# Autodesk Inventor assembly: Drive Tube Assem
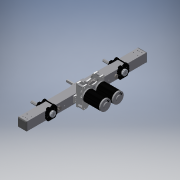
[picture p0: Inventor's stored thumbnail of the model, 180x180]
Saved by Autodesk Inventor 2019 (Build 230136000, 136)
## iProperties
Created: 2018-11-11
Part Number: Drive Tube Assem
Document SubType Name: Assembly
Designer: maste
Author: maste
## Documents named in this file (11)
- D:\Summer Drive Base V1\Summer Drivebase\Drive Tube Assem.iam
- D:\Summer Drive Base V1\Summer Drivebase\2x2 26in.ipt
- D:\Summer Drive Base V1\Summer Drivebase\Bearing Block Assem.iam
- D:\Summer Drive Base V1\Summer Drivebase\1in Spacer.ipt
- D:\Summer Drive Base V1\Summer Drivebase\0.0625in Spacer.ipt
- D:\Summer Drive Base V1\Summer Drivebase\36t_x_9mm_Wide_Double_Flange_Aluminum_Pulley_GT2_3mm_1_2_Hex_Bore_217-5873.ipt
- D:\Summer Drive Base V1\Summer Drivebase\Gearbox Assem.iam
- D:\Summer Drive Base V1\Summer Drivebase\Bearing Plate+Bearing.iam
- D:\Summer Drive Base V1\Summer Drivebase\0.125in Spacer.ipt
- D:\Summer Drive Base V1\Summer Drivebase\End Cap.ipt
- D:\Summer Drive Base V1\Summer Drivebase\217-3431-STEP.ipt
## Components (27 placed, 10 different names)
1. 2x2 26in:1 — Mate:1, Mate:2, Mate:3, Mate:4, Mate:5, Mate:6, Mate:27, Mate:28, Mate:29, Mate:30, Mate:31, Mate:32, Rotation:1, Mate:52, Mate:53, Mate:54, Mate:55, Mate:56, Mate:57, Mate:58, Mate:59, Rotation:2, Mate:60, Mate:61, Rotation:3
2. Bearing Block Assem:1 [sub-assembly] — Mate:4, Mate:5, Mate:6, Mate:7, Mate:8, Mate:9, Mate:14, Mate:17, Mate:18, Mate:20, Mate:21, Mate:43, Mate:44, Mate:45
3. Bearing Block Assem:2 [sub-assembly] — Mate:1, Mate:2, Mate:3, Mate:10, Mate:11, Mate:12, Mate:24, Mate:25, Mate:26, Mate:49, Mate:50, Mate:51
4. 1in Spacer:1 — Mate:10, Mate:11, Mate:12
5. 1in Spacer:2 — Mate:7, Mate:8, Mate:9, Mate:13, Mate:15
6. 0.0625in Spacer:1 — Mate:13, Mate:14, Mate:15, Mate:16
7. 0.0625in Spacer:2 — Mate:23, Flush:3, Flush:4
8. 36t_x_9mm_Wide_Double_Flange_Aluminum_Pulley_GT2_3mm_1_2_Hex_Bore_217-5873:1 — Mate:22, Flush:1, Flush:2, Mate:23, Flush:3, Flush:4
9. 36t_x_9mm_Wide_Double_Flange_Aluminum_Pulley_GT2_3mm_1_2_Hex_Bore_217-5873:2 — Mate:16, Mate:17, Mate:18, Mate:19
10. 0.0625in Spacer:3 — Mate:19, Mate:20, Mate:21
11. 0.0625in Spacer:4 — Mate:22, Flush:1, Flush:2, Mate:24, Mate:25, Mate:26
12. Gearbox Assem:1 [sub-assembly] — Mate:27, Mate:28, Mate:29, Mate:41, Mate:42, Mate:47, Mate:48
13. Bearing Plate+Bearing:1 [sub-assembly] — Mate:30, Mate:31, Mate:32, Rotation:1, Mate:40, Mate:46
14. 0.125in Spacer:1 — Mate:36, Flush:11, Flush:12, Mate:37, Flush:13, Flush:14
15. 0.125in Spacer:2 — Mate:35, Flush:9, Flush:10, Mate:36, Flush:11, Flush:12
16. 0.125in Spacer:3 — Mate:34, Flush:7, Flush:8, Mate:35, Flush:9, Flush:10
17. 36t_x_9mm_Wide_Double_Flange_Aluminum_Pulley_GT2_3mm_1_2_Hex_Bore_217-5873:3 — Mate:34, Flush:7, Flush:8, Mate:39, Flush:17, Flush:18
18. 36t_x_9mm_Wide_Double_Flange_Aluminum_Pulley_GT2_3mm_1_2_Hex_Bore_217-5873:4 — Mate:37, Flush:13, Flush:14, Mate:38, Flush:15, Flush:16
19. 0.125in Spacer:4 — Mate:39, Flush:17, Flush:18
20. 0.125in Spacer:5 — Mate:38, Flush:15, Flush:16, Mate:40, Mate:41, Mate:42
21. 0.0625in Spacer:5 — Mate:49, Mate:50, Mate:51
22. 0.0625in Spacer:6 — Mate:46, Mate:47, Mate:48
23. 0.0625in Spacer:7 — Mate:43, Mate:44, Mate:45
24. End Cap:1 — Mate:55, Mate:56, Mate:57
25. End Cap:2 — Mate:52, Mate:53, Mate:54
26. 217-3431-STEP:1 — Mate:60, Mate:61, Rotation:3
27. 217-3431-STEP:2 — Mate:58, Mate:59, Rotation:2
## Relationships (79: Mate 60, Flush 16, RelateRotation 3)
- Mate:1: 2x2 26in:1 ↔ Bearing Block Assem:2
- Mate:2: 2x2 26in:1 ↔ Bearing Block Assem:2
- Mate:3: 2x2 26in:1 ↔ Bearing Block Assem:2
- Mate:4: 2x2 26in:1 ↔ Bearing Block Assem:1
- Mate:5: 2x2 26in:1 ↔ Bearing Block Assem:1
- Mate:6: 2x2 26in:1 ↔ Bearing Block Assem:1
- Mate:7: Bearing Block Assem:1 ↔ 1in Spacer:2
- Mate:8: Bearing Block Assem:1 ↔ 1in Spacer:2
- Mate:9: Bearing Block Assem:1 ↔ 1in Spacer:2
- Mate:10: Bearing Block Assem:2 ↔ 1in Spacer:1
- Mate:11: Bearing Block Assem:2 ↔ 1in Spacer:1
- Mate:12: Bearing Block Assem:2 ↔ 1in Spacer:1
- Mate:13: 1in Spacer:2 ↔ 0.0625in Spacer:1
- Mate:14: Bearing Block Assem:1 ↔ 0.0625in Spacer:1
- Mate:15: 1in Spacer:2 ↔ 0.0625in Spacer:1
- Mate:16: 0.0625in Spacer:1 ↔ 36t_x_9mm_Wide_Double_Flange_Aluminum_Pulley_GT2_3mm_1_2_Hex_Bore_217-5873:2
- Mate:17: Bearing Block Assem:1 ↔ 36t_x_9mm_Wide_Double_Flange_Aluminum_Pulley_GT2_3mm_1_2_Hex_Bore_217-5873:2
- Mate:18: Bearing Block Assem:1 ↔ 36t_x_9mm_Wide_Double_Flange_Aluminum_Pulley_GT2_3mm_1_2_Hex_Bore_217-5873:2
- Mate:19: 36t_x_9mm_Wide_Double_Flange_Aluminum_Pulley_GT2_3mm_1_2_Hex_Bore_217-5873:2 ↔ 0.0625in Spacer:3
- Mate:20: Bearing Block Assem:1 ↔ 0.0625in Spacer:3
- Mate:21: Bearing Block Assem:1 ↔ 0.0625in Spacer:3
- Mate:22: 36t_x_9mm_Wide_Double_Flange_Aluminum_Pulley_GT2_3mm_1_2_Hex_Bore_217-5873:1 ↔ 0.0625in Spacer:4
- Flush:1: 36t_x_9mm_Wide_Double_Flange_Aluminum_Pulley_GT2_3mm_1_2_Hex_Bore_217-5873:1 ↔ 0.0625in Spacer:4
- Flush:2: 36t_x_9mm_Wide_Double_Flange_Aluminum_Pulley_GT2_3mm_1_2_Hex_Bore_217-5873:1 ↔ 0.0625in Spacer:4
- Mate:23: 0.0625in Spacer:2 ↔ 36t_x_9mm_Wide_Double_Flange_Aluminum_Pulley_GT2_3mm_1_2_Hex_Bore_217-5873:1
- Flush:3: 0.0625in Spacer:2 ↔ 36t_x_9mm_Wide_Double_Flange_Aluminum_Pulley_GT2_3mm_1_2_Hex_Bore_217-5873:1
- Flush:4: 0.0625in Spacer:2 ↔ 36t_x_9mm_Wide_Double_Flange_Aluminum_Pulley_GT2_3mm_1_2_Hex_Bore_217-5873:1
- Mate:24: Bearing Block Assem:2 ↔ 0.0625in Spacer:4
- Mate:25: Bearing Block Assem:2 ↔ 0.0625in Spacer:4
- Mate:26: Bearing Block Assem:2 ↔ 0.0625in Spacer:4
- Mate:27: 2x2 26in:1 ↔ Gearbox Assem:1
- Mate:28: 2x2 26in:1 ↔ Gearbox Assem:1
- Mate:29: 2x2 26in:1 ↔ Gearbox Assem:1
- Mate:30: 2x2 26in:1 ↔ Bearing Plate+Bearing:1
- Mate:31: 2x2 26in:1 ↔ Bearing Plate+Bearing:1
- Mate:32: 2x2 26in:1 ↔ Bearing Plate+Bearing:1
- Rotation:1 [RelateRotation] (1 ul): 2x2 26in:1 ↔ Bearing Plate+Bearing:1
- Mate:34: 0.125in Spacer:3 ↔ 36t_x_9mm_Wide_Double_Flange_Aluminum_Pulley_GT2_3mm_1_2_Hex_Bore_217-5873:3
- Flush:7: 0.125in Spacer:3 ↔ 36t_x_9mm_Wide_Double_Flange_Aluminum_Pulley_GT2_3mm_1_2_Hex_Bore_217-5873:3
- Flush:8: 0.125in Spacer:3 ↔ 36t_x_9mm_Wide_Double_Flange_Aluminum_Pulley_GT2_3mm_1_2_Hex_Bore_217-5873:3
- Mate:35: 0.125in Spacer:2 ↔ 0.125in Spacer:3
- Flush:9: 0.125in Spacer:2 ↔ 0.125in Spacer:3
- Flush:10: 0.125in Spacer:2 ↔ 0.125in Spacer:3
- Mate:36: 0.125in Spacer:1 ↔ 0.125in Spacer:2
- Flush:11: 0.125in Spacer:1 ↔ 0.125in Spacer:2
- Flush:12: 0.125in Spacer:1 ↔ 0.125in Spacer:2
- Mate:37: 0.125in Spacer:1 ↔ 36t_x_9mm_Wide_Double_Flange_Aluminum_Pulley_GT2_3mm_1_2_Hex_Bore_217-5873:4
- Flush:13: 0.125in Spacer:1 ↔ 36t_x_9mm_Wide_Double_Flange_Aluminum_Pulley_GT2_3mm_1_2_Hex_Bore_217-5873:4
- Flush:14: 0.125in Spacer:1 ↔ 36t_x_9mm_Wide_Double_Flange_Aluminum_Pulley_GT2_3mm_1_2_Hex_Bore_217-5873:4
- Mate:38: 36t_x_9mm_Wide_Double_Flange_Aluminum_Pulley_GT2_3mm_1_2_Hex_Bore_217-5873:4 ↔ 0.125in Spacer:5
- Flush:15: 36t_x_9mm_Wide_Double_Flange_Aluminum_Pulley_GT2_3mm_1_2_Hex_Bore_217-5873:4 ↔ 0.125in Spacer:5
- Flush:16: 36t_x_9mm_Wide_Double_Flange_Aluminum_Pulley_GT2_3mm_1_2_Hex_Bore_217-5873:4 ↔ 0.125in Spacer:5
- Mate:39: 36t_x_9mm_Wide_Double_Flange_Aluminum_Pulley_GT2_3mm_1_2_Hex_Bore_217-5873:3 ↔ 0.125in Spacer:4
- Flush:17: 36t_x_9mm_Wide_Double_Flange_Aluminum_Pulley_GT2_3mm_1_2_Hex_Bore_217-5873:3 ↔ 0.125in Spacer:4
- Flush:18: 36t_x_9mm_Wide_Double_Flange_Aluminum_Pulley_GT2_3mm_1_2_Hex_Bore_217-5873:3 ↔ 0.125in Spacer:4
- Mate:40: Bearing Plate+Bearing:1 ↔ 0.125in Spacer:5
- Mate:41: Gearbox Assem:1 ↔ 0.125in Spacer:5
- Mate:42: Gearbox Assem:1 ↔ 0.125in Spacer:5
- Mate:43: Bearing Block Assem:1 ↔ 0.0625in Spacer:7
- Mate:44: Bearing Block Assem:1 ↔ 0.0625in Spacer:7
- Mate:45: Bearing Block Assem:1 ↔ 0.0625in Spacer:7
- Mate:46: Bearing Plate+Bearing:1 ↔ 0.0625in Spacer:6
- Mate:47: Gearbox Assem:1 ↔ 0.0625in Spacer:6
- Mate:48: Gearbox Assem:1 ↔ 0.0625in Spacer:6
- Mate:49: Bearing Block Assem:2 ↔ 0.0625in Spacer:5
- Mate:50: Bearing Block Assem:2 ↔ 0.0625in Spacer:5
- Mate:51: Bearing Block Assem:2 ↔ 0.0625in Spacer:5
- Mate:52: 2x2 26in:1 ↔ End Cap:2
- Mate:53: 2x2 26in:1 ↔ End Cap:2
- Mate:54: 2x2 26in:1 ↔ End Cap:2
- Mate:55: 2x2 26in:1 ↔ End Cap:1
- Mate:56: 2x2 26in:1 ↔ End Cap:1
- Mate:57: 2x2 26in:1 ↔ End Cap:1
- Mate:58: 2x2 26in:1 ↔ 217-3431-STEP:2
- Mate:59: 2x2 26in:1 ↔ 217-3431-STEP:2
- Rotation:2 [RelateRotation] (1 ul): 2x2 26in:1 ↔ 217-3431-STEP:2
- Mate:60: 2x2 26in:1 ↔ 217-3431-STEP:1
- Mate:61: 2x2 26in:1 ↔ 217-3431-STEP:1
- Rotation:3 [RelateRotation] (1 ul): 2x2 26in:1 ↔ 217-3431-STEP:1
